# Autodesk Inventor assembly: Assemblysteun
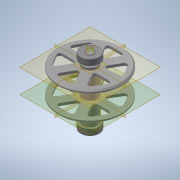
[picture p0: Inventor's stored thumbnail of the model, 180x180]
Saved by Autodesk Inventor 2021 (Build 250183000, 183)
## iProperties
Manager: PJ / DCS
Company: Emmaüs Bovenbouw Aalter
Created: 2021-03-01
Part Number: Assemblysteun
Catalog Web Link: http://emmausbovenbouw.op-weg.be/
Vendor: Emmaüs Bovenbouw Aalter
Document SubType Name: Assembly
Designer: Antho
Engineer: Declercq St.
Authority: Declercq St.
Title: Algemene Projecttitel
Author: Antho
## Documents named in this file (7)
- C:\Users\Antho\OneDrive\Documenten\Inventor\Inventor\GIP 6EM\Assembly\Steunwiel\Assemblysteun.iam
- C:\Users\Antho\OneDrive\Documenten\Inventor\Inventor\GIP 6EM\Wielen\Steunwiel\As.ipt
- C:\Users\Antho\OneDrive\Documenten\Inventor\Inventor\GIP 6EM\Wielen\Steunwiel\Hoes.ipt
- C:\Users\Antho\OneDrive\Documenten\Inventor\Inventor\GIP 6EM\Wielen\Steunwiel\Hoeswiel.ipt
- C:\Users\Antho\OneDrive\Documenten\Inventor\Inventor\GIP 6EM\Wielen\Steunwiel\Kleine Hoes.ipt
- C:\Users\Antho\OneDrive\Documenten\Inventor\Inventor\GIP 6EM\Wielen\Steunwiel\Wiel hout.ipt
- C:\Users\Antho\OneDrive\Documenten\Inventor\Inventor\GIP 6EM\Bevestigingen\Ball Bearing\W 619_6-2Z.iam
## Components (8 placed, 6 different names)
1. As:1 — Mate:1, Mate:2, Mate:5, Mate:6, Mate:8, Flush:1, Mate:10, Mate:12
2. Hoes:1 — Mate:6, Mate:7, Mate:9
3. Hoeswiel:1 — Mate:1, Mate:3, Mate:4
4. Kleine Hoes:1 — Mate:10, Mate:11
5. Wiel hout:1 — Mate:2, Mate:3, Mate:11
6. Wiel hout:2 — Mate:4, Mate:5, Mate:7
7. W 619_6-2Z:1 [sub-assembly] — Mate:8, Mate:9, Flush:1
8. W 619_6-2Z:2 [sub-assembly] — Mate:12
## Relationships (13: Mate 12, Flush 1)
- Mate:1: As:1 ↔ Hoeswiel:1
- Mate:2: As:1 ↔ Wiel hout:1
- Mate:3: Hoeswiel:1 ↔ Wiel hout:1
- Mate:4: Hoeswiel:1 ↔ Wiel hout:2
- Mate:5: As:1 ↔ Wiel hout:2
- Mate:6: As:1 ↔ Hoes:1
- Mate:7: Hoes:1 ↔ Wiel hout:2
- Mate:8: As:1 ↔ W 619_6-2Z:1
- Mate:9: Hoes:1 ↔ W 619_6-2Z:1
- Flush:1: As:1 ↔ W 619_6-2Z:1
- Mate:10: As:1 ↔ Kleine Hoes:1
- Mate:11: Kleine Hoes:1 ↔ Wiel hout:1
- Mate:12: As:1 ↔ W 619_6-2Z:2
